# Autodesk Inventor assembly: BasicDarthMaul
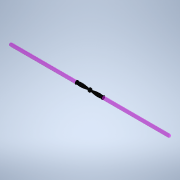
[picture p0: Inventor's stored thumbnail of the model, 180x180]
Saved by Autodesk Inventor 2021 (Build 250183000, 183)
## iProperties
Created: 2021-03-22
Part Number: BasicDarthMaul
Document SubType Name: Assembly
Designer: turnb
Author: turnb
## Documents named in this file (3)
- C:\Users\turnb\Documents\AutoDeskStuff\BasicDarthMaul.iam
- C:\Users\turnb\Documents\AutoDeskStuff\BasicHandle.ipt
- C:\Users\turnb\Documents\AutoDeskStuff\LightsaberBasicBladeButBad.ipt
## Components (4 placed, 2 different names)
1. BasicHandle:1 — Rotation:1
2. LightsaberBasicBladeButBad:1
3. BasicHandle:2 — Rotation:1, Rotation:2
4. LightsaberBasicBladeButBad:2 — Rotation:2
## Relationships (2: RevoluteJoint 2)
- Rotation:1 [RevoluteJoint]: BasicHandle:1 ↔ BasicHandle:2
- Rotation:2 [RevoluteJoint]: BasicHandle:2 ↔ LightsaberBasicBladeButBad:2
